# Autodesk Inventor assembly: robot
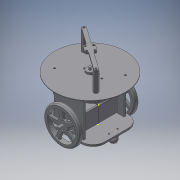
[picture p0: Inventor's stored thumbnail of the model, 180x180]
Saved by Autodesk Inventor 2017 (Build 210142000, 142)
## iProperties
Created: 2017-06-15
Part Number: robot
Document SubType Name: Assembly
Designer: millerid
Author: millerid
## Documents named in this file (13)
- U:\Research\Swarms\RobotModel\robot.iam
- U:\Research\Swarms\RobotModel\pcb.ipt
- U:\Research\Swarms\RobotModel\SG92R.ipt
- U:\Research\Swarms\RobotModel\NEMA11.ipt
- U:\Research\Swarms\RobotModel\halfincaster.ipt
- U:\Research\Swarms\RobotModel\1_5V_holder4AA.iam
- U:\Research\Swarms\RobotModel\Pololu 60mm Wheel.ipt
- U:\Research\Swarms\RobotModel\base_plate.ipt
- U:\Research\Swarms\RobotModel\side_plate.ipt
- U:\Research\Swarms\RobotModel\top_plate.ipt
- U:\Research\Swarms\RobotModel\quarterin_spacer.ipt
- U:\Research\Swarms\RobotModel\led_brace.ipt
- U:\Research\Swarms\RobotModel\oneandquarterstandoff.ipt
## Components (21 placed, 12 different names)
1. pcb:1 — Mate:1, Mate:2, Mate:21, Mate:24, Mate:25, Mate:27, Mate:28, Mate:29, Mate:30, Mate:33, Mate:34, Mate:35
2. SG92R:1 — Mate:1, Mate:2, Mate:21
3. NEMA11:1 — Mate:3, Mate:6, Mate:16, Mate:19
4. NEMA11:2 — Mate:5, Mate:14, Mate:15, Mate:20
5. halfincaster:1 — Mate:10, Mate:11
6. 1_5V_holder4AA:1 [sub-assembly] — Mate:7
7. Pololu 60mm Wheel:1 — Mate:3
8. halfincaster:2 — Mate:8, Mate:9
9. base_plate:1 — Mate:4, Mate:5, Mate:6, Mate:7, Mate:8, Mate:9, Mate:10, Mate:11, Mate:12, Mate:13, Mate:17, Mate:18, Mate:39
10. side_plate:1 — Mate:12, Mate:13, Mate:14, Mate:15, Mate:22, Mate:23
11. side_plate:2 — Mate:16, Mate:17, Mate:18, Mate:19
12. Pololu 60mm Wheel:2 — Mate:20
13. top_plate:1 — Mate:22, Mate:23, Mate:24, Mate:25, Mate:26
14. quarterin_spacer:1 — Mate:26, Mate:27
15. quarterin_spacer:2
16. quarterin_spacer:3 — Mate:28
17. quarterin_spacer:4 — Mate:29
18. quarterin_spacer:5 — Mate:30
19. led_brace:1 — Mate:36, Mate:37, Mate:38
20. oneandquarterstandoff:1 — Mate:33, Mate:34, Mate:36, Mate:37
21. oneandquarterstandoff:2 — Mate:35, Mate:38
## Relationships (37: Mate 37)
- Mate:1: pcb:1 ↔ SG92R:1
- Mate:2: pcb:1 ↔ SG92R:1
- Mate:3: NEMA11:1 ↔ Pololu 60mm Wheel:1
- Mate:4: base_plate:1
- Mate:5: NEMA11:2 ↔ base_plate:1
- Mate:6: NEMA11:1 ↔ base_plate:1
- Mate:7: 1_5V_holder4AA:1 ↔ base_plate:1
- Mate:8: halfincaster:2 ↔ base_plate:1
- Mate:9: halfincaster:2 ↔ base_plate:1
- Mate:10: halfincaster:1 ↔ base_plate:1
- Mate:11: halfincaster:1 ↔ base_plate:1
- Mate:12: base_plate:1 ↔ side_plate:1
- Mate:13: base_plate:1 ↔ side_plate:1
- Mate:14: NEMA11:2 ↔ side_plate:1
- Mate:15: NEMA11:2 ↔ side_plate:1
- Mate:16: NEMA11:1 ↔ side_plate:2
- Mate:17: base_plate:1 ↔ side_plate:2
- Mate:18: base_plate:1 ↔ side_plate:2
- Mate:19: NEMA11:1 ↔ side_plate:2
- Mate:20: NEMA11:2 ↔ Pololu 60mm Wheel:2
- Mate:21 (0.2 mm): pcb:1 ↔ SG92R:1
- Mate:22: side_plate:1 ↔ top_plate:1
- Mate:23: side_plate:1 ↔ top_plate:1
- Mate:24: pcb:1 ↔ top_plate:1
- Mate:25: pcb:1 ↔ top_plate:1
- Mate:26: top_plate:1 ↔ quarterin_spacer:1
- Mate:27: pcb:1 ↔ quarterin_spacer:1
- Mate:28: pcb:1 ↔ quarterin_spacer:3
- Mate:29: pcb:1 ↔ quarterin_spacer:4
- Mate:30: pcb:1 ↔ quarterin_spacer:5
- Mate:33: pcb:1 ↔ oneandquarterstandoff:1
- Mate:34: pcb:1 ↔ oneandquarterstandoff:1
- Mate:35: pcb:1 ↔ oneandquarterstandoff:2
- Mate:36: led_brace:1 ↔ oneandquarterstandoff:1
- Mate:37: led_brace:1 ↔ oneandquarterstandoff:1
- Mate:38 (0.1 mm): led_brace:1 ↔ oneandquarterstandoff:2
- Mate:39: base_plate:1
